# Autodesk Inventor assembly: Крепление мотора
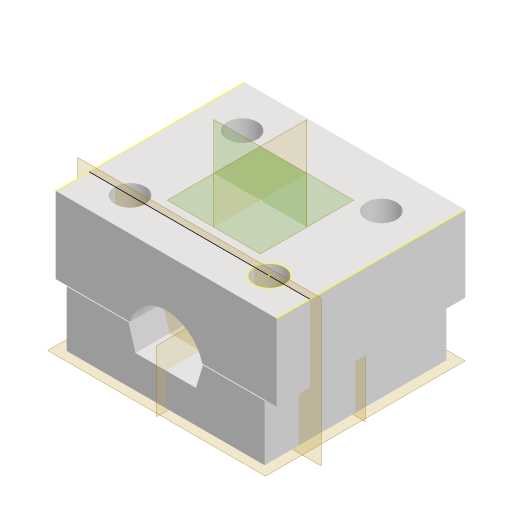
[picture p0: Inventor's stored thumbnail of the model, 512x512]
Saved by Autodesk Inventor 2023.2 (Build 272271030, 271C)
## iProperties
Created: 2024-12-18
Part Number: Крепление мотора
Document SubType Name: Assembly
Designer: I9232
Author: I9232
## Documents named in this file (3)
- D:\!Rover\Rover\Rover_construction\Крепление мотора.iam
- D:\!Rover\Rover\Rover_construction\Крепление мотора.ipt
- D:\!Rover\Rover\Rover_construction\Крепление мотора2.ipt
## Components (2 placed, 2 different names)
1. Нижняя часть крепления мотора:1 — Совмещение:1, Совмещение:2, Совмещение:3
2. Крепление мотора2:1 — Совмещение:1, Совмещение:2, Угол:1
## Relationships (4: Mate 3, Angle 1)
- Совмещение:1 [Mate]: Нижняя часть крепления мотора:1 ↔ Крепление мотора2:1
- Совмещение:2 [Mate]: Нижняя часть крепления мотора:1 ↔ Крепление мотора2:1
- Совмещение:3 [Mate]: Нижняя часть крепления мотора:1
- Угол:1 [Angle] (90 deg): Крепление мотора2:1
